# Autodesk Inventor assembly: 6P Sprocket
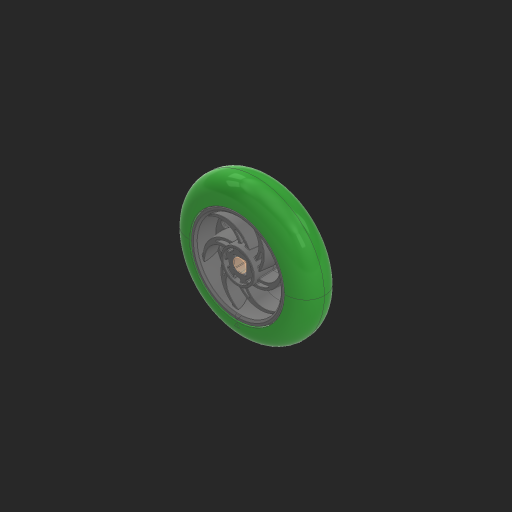
[picture p0: Inventor's stored thumbnail of the model, 512x512]
Saved by Autodesk Inventor 2023 (Build 270158000, 158)
## iProperties
Created: 2022-08-02
Part Number: 6P Sprocket
Document SubType Name: Assembly
Designer: ylu12
Author: ylu12
## Documents named in this file (23)
- C:\Users\ylu12\Documents\GitHub\VEX-CAD-Inventor\Motion\Wheels\Traction Wheel.iam
- C:\Users\ylu12\Documents\GitHub\VEX-CAD-Inventor\Motion\HS Shaft Adapter Circle.ipt
- C:\Users\ylu12\Documents\GitHub\VEX-CAD-Inventor\Motion\HS Shaft Adapter Square.ipt
- C:\Users\ylu12\Documents\GitHub\VEX-CAD-Inventor\Motion\Wheels\Reference Files\2.75 Traction, No Insert.ipt
- C:\Users\ylu12\Documents\GitHub\VEX-CAD-Inventor\Motion\Wheels\Reference Files\3.25 Traction, No Insert.ipt
- C:\Users\ylu12\Documents\GitHub\VEX-CAD-Inventor\Motion\Wheels\Reference Files\4 Omni Locked, No Insert.ipt
- C:\Users\ylu12\Documents\GitHub\VEX-CAD-Inventor\Motion\Wheels\Reference Files\4 Traction, No Insert.ipt
- C:\Users\ylu12\Documents\GitHub\VEX-CAD-Inventor\Motion\Wheels\Reference Files\169 Traction, No Insert.ipt
- 169 Traction, Circle.iam
- 169 Traction, No Insert.iam
- 169 Traction, Square.iam
- 2.75 Traction, Circle.iam
- 2.75 Traction, No Insert.iam
- 2.75 Traction, Square.iam
- 3.25 Traction, Circle.iam
- 3.25 Traction, No Insert.iam
- 3.25 Traction, Square.iam
- 4 Omni Locked, Circle.iam
- 4 Omni Locked, No Insert.iam
- 4 Omni Locked, Square.iam
- 4 Traction, Circle.iam
- 4 Traction, No Insert.iam
- 4 Traction, Square.iam
## Components (7 placed, 7 different names)
1. Circle — Flush:1, Mate:1, Mate:3
2. Square — Flush:2, Mate:2, Mate:4
3. 2.75 Traction — Mate:5, Mate:6, Flush:3
4. 3.25 Traction — Flush:4, Mate:7, Mate:8
5. 4 Omni Locked — Flush:5, Mate:9, Mate:10
6. 4 Traction — Flush:6, Mate:11, Mate:12
7. 169 Traction — Flush:7, Mate:13, Mate:14
## Relationships (21: Mate 14, Flush 7)
- Flush:1 (6.35 mm): Circle
- Flush:2 (6.35 mm): Square
- Mate:1: Circle
- Mate:2: Square
- Mate:3: Circle
- Mate:4: Square
- Mate:5: 2.75 Traction
- Mate:6: 2.75 Traction
- Flush:3: 2.75 Traction
- Flush:4: 3.25 Traction
- Flush:5: 4 Omni Locked
- Flush:6: 4 Traction
- Flush:7: 169 Traction
- Mate:7: 3.25 Traction
- Mate:8: 3.25 Traction
- Mate:9: 4 Omni Locked
- Mate:10: 4 Omni Locked
- Mate:11: 4 Traction
- Mate:12: 4 Traction
- Mate:13: 169 Traction
- Mate:14: 169 Traction
